# Autodesk Inventor assembly: Assembly1
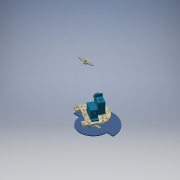
[picture p0: Inventor's stored thumbnail of the model, 180x180]
Saved by Autodesk Inventor 2017 (Build 210142000, 142)
## iProperties
Created: 2016-12-07
Part Number: Assembly1
Document SubType Name: Assembly
Designer: PLTW
Author: PLTW
## Documents named in this file (5)
- C:\Users\PLTW\Documents\Inventor\FIRSTStuff\Assembly1.iam
- C:\Users\PLTW\Documents\Inventor\FIRSTStuff\PixyCamGimbal Base.ipt
- C:\Users\PLTW\Documents\Inventor\FIRSTStuff\PixyCamGimbal Body.ipt
- C:\Users\PLTW\Documents\Inventor\FIRSTStuff\servo body.ipt
- C:\Users\PLTW\Documents\Inventor\FIRSTStuff\Servo Horn.ipt
## Components (6 placed, 4 different names)
1. PixyCamGimbal Base:1 — Insert:1, Angle:1
2. PixyCamGimbal Body:1 — Mate:1, Mate:2, Mate:3, Mate:4, Mate:5, Mate:6
3. servo body:1 — Mate:4, Mate:5, Mate:6
4. Servo Horn:1
5. Servo Horn:2 — Insert:1, Angle:1, Insert:2
6. servo body:2 — Insert:2, Mate:1, Mate:2, Mate:3
## Relationships (9: Mate 6, Insert 2, Angle 1)
- Insert:1: PixyCamGimbal Base:1 ↔ Servo Horn:2
- Angle:1 (0 deg): PixyCamGimbal Base:1 ↔ Servo Horn:2
- Insert:2: Servo Horn:2 ↔ servo body:2
- Mate:1: PixyCamGimbal Body:1 ↔ servo body:2
- Mate:2: PixyCamGimbal Body:1 ↔ servo body:2
- Mate:3: PixyCamGimbal Body:1 ↔ servo body:2
- Mate:4: PixyCamGimbal Body:1 ↔ servo body:1
- Mate:5: PixyCamGimbal Body:1 ↔ servo body:1
- Mate:6: PixyCamGimbal Body:1 ↔ servo body:1
